# Autodesk Inventor assembly: assembled
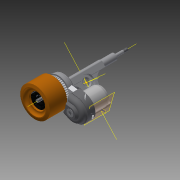
[picture p0: Inventor's stored thumbnail of the model, 180x180]
Saved by Autodesk Inventor 2015 SP1 (Build 190203100, 203)
## iProperties
Created: 2014-11-17
Part Number: assembled
Document SubType Name: Assembly
Designer: brent
Author: brent
## Documents named in this file (10)
- C:\Users\brent\Documents\electric-longboard\brent2\assembled.iam
- C:\Users\brent\Documents\electric-longboard\brent2\50cal.iam
- C:\Users\brent\Documents\electric-longboard\brent2\mount.iam
- C:\Users\brent\Documents\electric-longboard\brent2\mount_alt.ipt
- C:\Users\brent\Documents\electricskateboard\MotorAssembly.iam
- C:\Users\brent\Documents\electric-longboard\brent\Imported Components\15t_pulley\15t_pulley.ipt
- C:\Users\brent\Documents\electric-longboard\brent2\pulley_cover.ipt
- C:\Users\brent\Documents\electric-longboard\dliu\Board\Wheel Blank Pro 83mm.ipt
- C:\Users\brent\Documents\electric-longboard\brent2\pulley_protector_alt.ipt
- C:\Users\brent\Documents\electric-longboard\brent\wheelinsertinner40t.ipt
## Components (9 placed, 9 different names)
1. 50cal:1 [sub-assembly] — Mate:1, Mate:2, Mate:3, Mate:4, Mate:14, Mate:19, Mate:22
2. mount:1 [sub-assembly] — Mate:1, Mate:2
3. mount_alt:1 — Mate:3, Mate:4, Mate:5, Mate:6, Mate:10, Mate:11, Mate:12, Mate:13, Mate:15, Mate:18, Mate:20, Mate:21
4. MotorAssembly:1 [sub-assembly] — Mate:5, Mate:6, Mate:9, Mate:13, Mate:18
5. 15t_pulley:1 — Mate:9
6. pulley_cover:1 — Mate:10, Mate:11, Mate:12, Mate:15, Mate:16, Mate:17
7. Wheel Blank Pro 83mm:1 — Mate:14, Mate:16, Mate:17
8. pulley_protector_alt:1 — Mate:19, Mate:20, Mate:21
9. wheelinsertinner40t:1 — Mate:22
## Relationships (20: Mate 20)
- Mate:1: 50cal:1 ↔ mount:1
- Mate:2: 50cal:1 ↔ mount:1
- Mate:3: 50cal:1 ↔ mount_alt:1
- Mate:4 (1.27 mm): 50cal:1 ↔ mount_alt:1
- Mate:5: mount_alt:1 ↔ MotorAssembly:1
- Mate:6: mount_alt:1 ↔ MotorAssembly:1
- Mate:9: MotorAssembly:1 ↔ 15t_pulley:1
- Mate:10: mount_alt:1 ↔ pulley_cover:1
- Mate:11: mount_alt:1 ↔ pulley_cover:1
- Mate:12: mount_alt:1 ↔ pulley_cover:1
- Mate:13: mount_alt:1 ↔ MotorAssembly:1
- Mate:14: 50cal:1 ↔ Wheel Blank Pro 83mm:1
- Mate:15: mount_alt:1 ↔ pulley_cover:1
- Mate:16: pulley_cover:1 ↔ Wheel Blank Pro 83mm:1
- Mate:17: pulley_cover:1 ↔ Wheel Blank Pro 83mm:1
- Mate:18: mount_alt:1 ↔ MotorAssembly:1
- Mate:19: 50cal:1 ↔ pulley_protector_alt:1
- Mate:20: mount_alt:1 ↔ pulley_protector_alt:1
- Mate:21: mount_alt:1 ↔ pulley_protector_alt:1
- Mate:22: 50cal:1 ↔ wheelinsertinner40t:1
